# Autodesk Inventor assembly: PARA IMAGEN PPAL
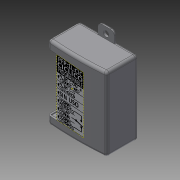
[picture p0: Inventor's stored thumbnail of the model, 180x180]
Saved by Autodesk Inventor 2013 (Build 170138000, 138)
## iProperties
Created: 2018-10-18
Part Number: PARA IMAGEN PPAL
Document SubType Name: Assembly
Designer: Fede
Author: Fede
## Documents named in this file (6)
- J:\0000 FEDE\16GB\0000 INTERIOR\DE_TMP_1L\MANUALES\0000_IMG\3d\PARA IMAGEN PPAL.iam
- J:\0000 FEDE\16GB\0000 INTERIOR\DE_TMP_1L\MANUALES\0000_IMG\3d\cuerpo.ipt
- J:\0000 FEDE\16GB\0000 INTERIOR\DE_TMP_1L\MANUALES\0000_IMG\3d\tapa.ipt
- J:\0000 FEDE\256GB\inventor\FILTRO\Imported Components\TMP_1L\TMP_1L.iam
- J:\0000 FEDE\16GB\0000 INTERIOR\DE_TMP_1L\MANUALES\0000_IMG\3d\E_BORNERA.ipt
- J:\0000 FEDE\16GB\0000 INTERIOR\DE_TMP_1L\MANUALES\0000_IMG\3d\E_ET.ipt
## Components (5 placed, 5 different names)
1. cuerpo:1 — Mate:1, Flush:1, Flush:2, Mate:4
2. tapa:1 — Mate:1, Flush:1, Flush:2, Mate:3, Flush:3
3. TMP_1L:2 [sub-assembly] — Mate:3, Flush:3, Mate:5
4. E_BORNERA:1 — Mate:5
5. E_ET:1 — Mate:4
## Relationships (7: Mate 4, Flush 3)
- Mate:1: cuerpo:1 ↔ tapa:1
- Flush:1: cuerpo:1 ↔ tapa:1
- Flush:2: cuerpo:1 ↔ tapa:1
- Mate:3: tapa:1 ↔ TMP_1L:2
- Flush:3 (0.5 mm): tapa:1 ↔ TMP_1L:2
- Mate:4: cuerpo:1 ↔ E_ET:1
- Mate:5: TMP_1L:2 ↔ E_BORNERA:1
